# Autodesk Inventor assembly: OBUDOWA PRZEDNIA + PRZYCISKI + MATRYCA
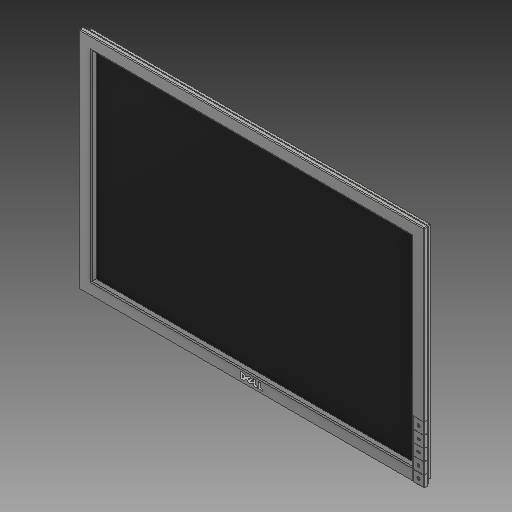
[picture p0: Inventor's stored thumbnail of the model, 512x512]
Saved by Autodesk Inventor 2017 SP1 (Build 210196100, 196)
## iProperties
Created: 2021-03-07
Part Number: OBUDOWA PRZEDNIA + PRZYCISKI + MATRYCA
Document SubType Name: Assembly
Designer: Administrator
Author: Administrator
## Documents named in this file (8)
- D:\PRYWATNE\PROJEKTY\POKÓJ\URZĄDZENIA PERYFERYJNE\DELL 1909Wf\OBUDOWA PRZEDNIA + PRZYCISKI + MATRYCA.iam
- D:\PRYWATNE\PROJEKTY\POKÓJ\URZĄDZENIA PERYFERYJNE\DELL 1909Wf\OBUDOWA PRZEDNIA.ipt
- D:\PRYWATNE\PROJEKTY\POKÓJ\URZĄDZENIA PERYFERYJNE\DELL 1909Wf\PRZYCISK IO.ipt
- D:\PRYWATNE\PROJEKTY\POKÓJ\URZĄDZENIA PERYFERYJNE\DELL 1909Wf\PRZYCISK MENU.ipt
- D:\PRYWATNE\PROJEKTY\POKÓJ\URZĄDZENIA PERYFERYJNE\DELL 1909Wf\PRZYCISK AUTO ADJUST.ipt
- D:\PRYWATNE\PROJEKTY\POKÓJ\URZĄDZENIA PERYFERYJNE\DELL 1909Wf\PRZYCISK INPUT SOURCE .ipt
- D:\PRYWATNE\PROJEKTY\POKÓJ\URZĄDZENIA PERYFERYJNE\DELL 1909Wf\PRZYCISK BRIGTNESS_CONTRAST.ipt
- D:\PRYWATNE\PROJEKTY\POKÓJ\URZĄDZENIA PERYFERYJNE\DELL 1909Wf\MATRYCA.ipt
## Components (7 placed, 7 different names)
1. OBUDOWA PRZEDNIA:1 — Równoległy:1, Zestawiający:1, Równoległy:2, Zestawiający:2, Zestawiający:5, Zestawiający:7, Zestawiający:9, Równoległy:7, Zestawiający:13, Zestawiający:14
2. PRZYCISK BRIGTNESS_CONTRAST:1 — Zestawiający:9, Zestawiający:12, Równoległy:10
3. PRZYCISK AUTO ADJUST:1 — Zestawiający:5, Zestawiający:11, Równoległy:9, Zestawiający:12, Równoległy:10
4. PRZYCISK INPUT SOURCE :1 — Zestawiający:7, Zestawiający:10, Równoległy:8, Zestawiający:11, Równoległy:9
5. PRZYCISK MENU:1 — Zestawiający:1, Równoległy:3, Zestawiający:3, Zestawiający:10, Równoległy:8
6. PRZYCISK IO:1 — Równoległy:1, Równoległy:2, Równoległy:3, Zestawiający:2, Zestawiający:3
7. MATRYCA:1 — Równoległy:7, Zestawiający:13, Zestawiający:14
## Relationships (18: Mate 11, Flush 7)
- Równoległy:1 [Flush]: OBUDOWA PRZEDNIA:1 ↔ PRZYCISK IO:1
- Zestawiający:1 [Mate] (0.25 mm): OBUDOWA PRZEDNIA:1 ↔ PRZYCISK MENU:1
- Równoległy:2 [Flush]: OBUDOWA PRZEDNIA:1 ↔ PRZYCISK IO:1
- Równoległy:3 [Flush]: PRZYCISK MENU:1 ↔ PRZYCISK IO:1
- Zestawiający:2 [Mate] (0.25 mm): OBUDOWA PRZEDNIA:1 ↔ PRZYCISK IO:1
- Zestawiający:3 [Mate] (0.25 mm): PRZYCISK MENU:1 ↔ PRZYCISK IO:1
- Zestawiający:5 [Mate] (0.25 mm): OBUDOWA PRZEDNIA:1 ↔ PRZYCISK AUTO ADJUST:1
- Zestawiający:7 [Mate] (0.25 mm): OBUDOWA PRZEDNIA:1 ↔ PRZYCISK INPUT SOURCE :1
- Zestawiający:9 [Mate] (0.25 mm): OBUDOWA PRZEDNIA:1 ↔ PRZYCISK BRIGTNESS_CONTRAST:1
- Równoległy:7 [Flush]: OBUDOWA PRZEDNIA:1 ↔ MATRYCA:1
- Zestawiający:10 [Mate] (0.25 mm): PRZYCISK INPUT SOURCE :1 ↔ PRZYCISK MENU:1
- Równoległy:8 [Flush]: PRZYCISK INPUT SOURCE :1 ↔ PRZYCISK MENU:1
- Zestawiający:11 [Mate] (0.25 mm): PRZYCISK AUTO ADJUST:1 ↔ PRZYCISK INPUT SOURCE :1
- Równoległy:9 [Flush]: PRZYCISK AUTO ADJUST:1 ↔ PRZYCISK INPUT SOURCE :1
- Zestawiający:12 [Mate] (0.25 mm): PRZYCISK BRIGTNESS_CONTRAST:1 ↔ PRZYCISK AUTO ADJUST:1
- Równoległy:10 [Flush]: PRZYCISK BRIGTNESS_CONTRAST:1 ↔ PRZYCISK AUTO ADJUST:1
- Zestawiający:13 [Mate] (5.5 mm): OBUDOWA PRZEDNIA:1 ↔ MATRYCA:1
- Zestawiający:14 [Mate] (4.269 mm): OBUDOWA PRZEDNIA:1 ↔ MATRYCA:1
